# Autodesk Inventor assembly: sus1
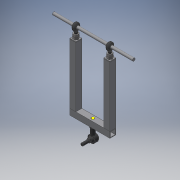
[picture p0: Inventor's stored thumbnail of the model, 180x180]
Saved by Autodesk Inventor 2018 (Build 220112000, 112)
## iProperties
Created: 2017-09-08
Part Number: sus1
Material: 一般
Document SubType Name: Assembly
Designer: mura5
Author: mura5
## Documents named in this file (7)
- C:\Users\mura5\Documents\RBBR\cart\A.iam
- C:\Users\mura5\Documents\RBBR\cart\Rod1.iam
- C:\Users\mura5\Documents\RBBR\cart\iko_POS_14EC\AIS2016\POS 14ECBall.ipt
- C:\Users\mura5\Documents\RBBR\cart\Shaft14mm.ipt
- C:\Users\mura5\Documents\RBBR\cart\iko_LHSA_14\AIS2016\LHSA 14 Body1.ipt
- C:\Users\mura5\Documents\RBBR\cart\iko_LHSA_14\AIS2016\LHSA 14 Body2.ipt
- C:\Users\mura5\Documents\RBBR\cart\Pipe3.ipt
## Components (8 placed, 6 different names)
1. POS 14ECBall:1 — 回転:1, 円柱状:1, メイト:9, ボール:4
2. Rod1:1 [sub-assembly] — リジッド:2, ボール:4
3. Rod1:2 [sub-assembly] — ボール:2, リジッド:1
4. POS 14ECBall:2 — ボール:2, 回転:1, 円柱状:2, メイト:9
5. Shaft14mm:1 — 円柱状:1, 円柱状:2
6. LHSA 14 Body1:1 — ボール:3, リジッド:3
7. LHSA 14 Body2:1 — ボール:3
8. Pipe3:1 — リジッド:1, リジッド:2, リジッド:3
## Relationships (10: BallJoint 3, WeldJoint 3, CylindricalJoint 2, RevoluteJoint 1, Mate 1)
- ボール:2 [BallJoint]: Rod1:2 ↔ POS 14ECBall:2
- 回転:1 [RevoluteJoint] (200 mm): POS 14ECBall:1 ↔ POS 14ECBall:2
- 円柱状:1 [CylindricalJoint]: POS 14ECBall:1 ↔ Shaft14mm:1
- 円柱状:2 [CylindricalJoint]: POS 14ECBall:2 ↔ Shaft14mm:1
- ボール:3 [BallJoint]: LHSA 14 Body1:1 ↔ LHSA 14 Body2:1
- メイト:9 [Mate] (200 mm): POS 14ECBall:1 ↔ POS 14ECBall:2
- リジッド:1 [WeldJoint]: Rod1:2 ↔ Pipe3:1
- リジッド:2 [WeldJoint]: Rod1:1 ↔ Pipe3:1
- ボール:4 [BallJoint]: POS 14ECBall:1 ↔ Rod1:1
- リジッド:3 [WeldJoint]: LHSA 14 Body1:1 ↔ Pipe3:1
